# Autodesk Inventor assembly: LED Structure Assembly
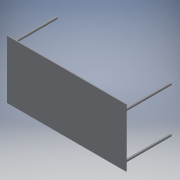
[picture p0: Inventor's stored thumbnail of the model, 180x180]
Saved by Autodesk Inventor 2017 (Build 210142000, 142)
## iProperties
Created: 2017-01-06
Part Number: LED Structure Assembly
Document SubType Name: Assembly
Designer: umr
Author: umr
## Documents named in this file (4)
- D:\SeniorProject\Models2\LED Structure\LED Structure Assembly.iam
- D:\SeniorProject\Models2\LED Tube\lampara 54 leds.iam
- D:\SeniorProject\Models2\LED Structure\Led Plater.ipt
- D:\SeniorProject\Models2\LED Structure\Support.ipt
## Components (15 placed, 3 different names)
1. Led Plater:1 — Mate:1, Mate:2, Mate:3, Mate:4, Mate:5, Mate:6, Mate:7, Mate:8, Mate:9
2. Support:1 — Mate:2, Mate:3
3. Support:2 — Mate:4, Mate:7
4. Support:3 — Mate:6, Mate:8
5. Support:4 — Mate:5, Mate:9
6. lampara 54 leds:1 [sub-assembly] — Mate:1
7. lampara 54 leds:2 [sub-assembly]
8. lampara 54 leds:3 [sub-assembly]
9. lampara 54 leds:4 [sub-assembly]
10. lampara 54 leds:5 [sub-assembly]
11. lampara 54 leds:6 [sub-assembly]
12. lampara 54 leds:7 [sub-assembly]
13. lampara 54 leds:8 [sub-assembly]
14. lampara 54 leds:9 [sub-assembly]
15. lampara 54 leds:10 [sub-assembly]
## Component patterns: (10 elements, first: lampara 54 leds:1)
## Relationships (9: Mate 9)
- Mate:1: Led Plater:1 ↔ lampara 54 leds:1
- Mate:2: Led Plater:1 ↔ Support:1
- Mate:3: Led Plater:1 ↔ Support:1
- Mate:4: Led Plater:1 ↔ Support:2
- Mate:5: Led Plater:1 ↔ Support:4
- Mate:6: Led Plater:1 ↔ Support:3
- Mate:7: Led Plater:1 ↔ Support:2
- Mate:8: Led Plater:1 ↔ Support:3
- Mate:9: Led Plater:1 ↔ Support:4
